# Autodesk Inventor assembly: nozzle
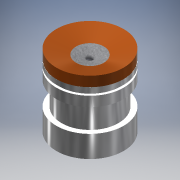
[picture p0: Inventor's stored thumbnail of the model, 180x180]
Saved by Autodesk Inventor 2017 (Build 210142000, 142)
## iProperties
Created: 2016-10-19
Part Number: nozzle
Document SubType Name: Assembly
Designer: cflannery
Author: cflannery
## Documents named in this file (7)
- D:\Triton_Rocket_Club\Propulsion\Users\cflannery\candy_rocket\nozzle.iam
- D:\Triton_Rocket_Club\Propulsion\Users\cflannery\candy_rocket\aluminum_carrier.ipt
- D:\Triton_Rocket_Club\Propulsion\Users\cflannery\candy_rocket\aluminum_retainer.ipt
- D:\Triton_Rocket_Club\Propulsion\Users\cflannery\candy_rocket\aluminum_skirt.ipt
- D:\Triton_Rocket_Club\Propulsion\Users\cflannery\candy_rocket\graphite.ipt
- D:\Triton_Rocket_Club\Propulsion\Users\cflannery\candy_rocket\phenolic_cap.ipt
- D:\Triton_Rocket_Club\Propulsion\Users\cflannery\candy_rocket\phenolic_liner.ipt
## Components (6 placed, 6 different names)
1. aluminum_carrier:1 — Mate:5, Mate:6, Mate:7, Mate:8, Mate:9, Mate:10
2. aluminum_retainer:1 — Mate:7, Mate:9
3. aluminum_skirt:1 — Mate:6, Mate:10
4. graphite:1 — Mate:1, Mate:2, Mate:3, Mate:4
5. phenolic_cap:1 — Mate:1, Mate:2, Mate:8
6. phenolic_liner:1 — Mate:3, Mate:4, Mate:5
## Relationships (10: Mate 10)
- Mate:1: graphite:1 ↔ phenolic_cap:1
- Mate:2: graphite:1 ↔ phenolic_cap:1
- Mate:3: graphite:1 ↔ phenolic_liner:1
- Mate:4: graphite:1 ↔ phenolic_liner:1
- Mate:5: aluminum_carrier:1 ↔ phenolic_liner:1
- Mate:6: aluminum_carrier:1 ↔ aluminum_skirt:1
- Mate:7: aluminum_carrier:1 ↔ aluminum_retainer:1
- Mate:8: aluminum_carrier:1 ↔ phenolic_cap:1
- Mate:9: aluminum_carrier:1 ↔ aluminum_retainer:1
- Mate:10: aluminum_carrier:1 ↔ aluminum_skirt:1
